# Autodesk Inventor assembly: Assembly1
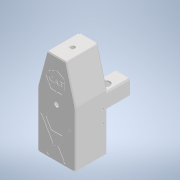
[picture p0: Inventor's stored thumbnail of the model, 180x180]
Saved by Autodesk Inventor 2022 (Build 260153000, 153)
## iProperties
Created: 2023-01-18
Part Number: Assembly1
Document SubType Name: Assembly
Designer: chris
Author: chris
## Documents named in this file (5)
- C:\Users\chris\Desktop\STL files\CAT\Assembly1.iam
- C:\Users\chris\Desktop\STL files\CAT\the box.ipt
- C:\Users\chris\Desktop\STL files\CAT\the box cover.ipt
- C:\Users\chris\Desktop\STL files\CAT\the handle.ipt
- C:\Users\chris\Desktop\STL files\CAT\bottom_cap_handle.ipt
## Components (4 placed, 4 different names)
1. the box:1 — Rotational:1, Flush:1, Rotational:2, Mate:1
2. the handle:1 — Rotational:2, Mate:1, Rotational:3, Mate:2
3. bottom_cap_handle:1 — Rotational:3, Mate:2
4. the box cover:1 — Rotational:1, Flush:1
## Relationships (6: RevoluteJoint 3, Mate 2, Flush 1)
- Rotational:1 [RevoluteJoint]: the box:1 ↔ the box cover:1
- Flush:1: the box:1 ↔ the box cover:1
- Rotational:2 [RevoluteJoint]: the box:1 ↔ the handle:1
- Mate:1: the box:1 ↔ the handle:1
- Rotational:3 [RevoluteJoint]: the handle:1 ↔ bottom_cap_handle:1
- Mate:2: the handle:1 ↔ bottom_cap_handle:1
